# Autodesk Inventor assembly: Blue Alliance Arm
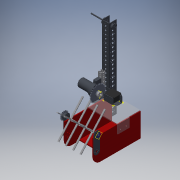
[picture p0: Inventor's stored thumbnail of the model, 180x180]
Saved by Autodesk Inventor 2016 (Build 200138000, 138)
## iProperties
Created: 2015-12-20
Part Number: Blue Alliance Arm
Document SubType Name: Assembly
Designer: tbloo
Author: tbloo
## Documents named in this file (14)
- C:\Users\TimB\Documents\GitHub\phi_robotics\3d-models\FTC_Tetrix_KOP_Block_Party\Tim Bloot Designs\JAr JaR Bot\Red Alliance Arm.iam
- C:\Users\TimB\Documents\GitHub\phi_robotics\3d-models\FTC_Tetrix_KOP_Block_Party\Tetrix_Kit_FTC\Autodesk Inventor Files\tetrix_axle.ipt
- C:\Users\TimB\Documents\GitHub\phi_robotics\3d-models\FTC_Tetrix_KOP_Block_Party\Tetrix_Kit_FTC\Autodesk Inventor Files\tetrix_axle_lock.iam
- C:\Users\TimB\Documents\GitHub\phi_robotics\3d-models\FTC_Tetrix_KOP_Block_Party\Tetrix_Kit_FTC\Autodesk Inventor Files\tetrix_c_channel-1.ipt
- C:\Users\TimB\Documents\GitHub\phi_robotics\3d-models\FTC_Tetrix_KOP_Block_Party\Tim Bloot Designs\JAr JaR Bot\cube channel short.ipt
- C:\Users\TimB\Documents\GitHub\phi_robotics\3d-models\FTC_Tetrix_KOP_Block_Party\Tetrix_Kit_FTC\Autodesk Inventor Files\tetrix_motor_mount-old.ipt
- C:\Users\TimB\Documents\GitHub\phi_robotics\3d-models\FTC_Tetrix_KOP_Block_Party\Tetrix_Kit_FTC\Autodesk Inventor Files\tetrix_motor.iam
- C:\Users\TimB\Documents\GitHub\phi_robotics\3d-models\FTC_Tetrix_KOP_Block_Party\Tetrix_Kit_FTC\Autodesk Inventor Files\tetrix_maxle_lock.iam
- C:\Users\TimB\Documents\GitHub\phi_robotics\3d-models\FTC_Tetrix_KOP_Block_Party\Tetrix_Kit_FTC\Autodesk Inventor Files\tetrix_chain_gear-32t.ipt
- C:\Users\TimB\Documents\GitHub\phi_robotics\3d-models\FTC_Tetrix_KOP_Block_Party\Tetrix_Kit_FTC\Autodesk Inventor Files\tetrix_screw.ipt
- C:\Users\TimB\Documents\GitHub\phi_robotics\3d-models\FTC_Tetrix_KOP_Block_Party\Tim Bloot Designs\JAr JaR Bot\Red Alliance Bucket.iam
- C:\Users\TimB\Documents\GitHub\phi_robotics\3d-models\FTC_Tetrix_KOP_Block_Party\Tetrix_Kit_FTC\Autodesk Inventor Files\tetrix_Lbracket-round.ipt
- C:\Users\TimB\Documents\GitHub\phi_robotics\3d-models\FTC_Tetrix_KOP_Block_Party\Tetrix_Kit_FTC\Autodesk Inventor Files\tetrix_c_channel-round.ipt
- C:\Users\TimB\Documents\GitHub\phi_robotics\3d-models\FTC_Tetrix_KOP_Block_Party\Tim Bloot Designs\JAr JaR Bot\cut c channel.ipt
## Components (16 placed, 13 different names)
1. tetrix_axle:1 — Rigid:1
2. tetrix_axle_lock:1 [sub-assembly] — Rigid:16
3. tetrix_axle_lock:2 [sub-assembly] — Rigid:1, Rigid:15
4. tetrix_c_channel-1:1 — Rigid:19
5. tetrix_c_channel-1:2 — Mate:1, Flush:1, Flush:2, Rigid:20
6. cube channel short:1 — Rigid:12, Rigid:17
7. tetrix_motor_mount-old:1 — Rigid:12, Rotational:1
8. tetrix_motor:1 [sub-assembly] — Rigid:11, Rotational:1
9. tetrix_maxle_lock:1 [sub-assembly] — Rigid:8, Rigid:11
10. tetrix_chain_gear-32t:1 — Rigid:8, Rigid:9, Rigid:10
11. tetrix_screw:1 — Rigid:10
12. tetrix_screw:2 — Rigid:9
13. Red Alliance Bucket:1 [sub-assembly] — Mate:1, Flush:1, Flush:2
14. tetrix_Lbracket-round:1 — Rigid:14, Rigid:18
15. tetrix_c_channel-round:1 — Rigid:14
16. cut c channel:1 — Rigid:15, Rigid:16, Rigid:17, Rigid:18, Rigid:19, Rigid:20
## Relationships (17: WeldJoint 13, Flush 2, RevoluteJoint 1, Mate 1)
- Rigid:1 [WeldJoint]: tetrix_axle:1 ↔ tetrix_axle_lock:2
- Rigid:8 [WeldJoint]: tetrix_maxle_lock:1 ↔ tetrix_chain_gear-32t:1
- Rigid:9 [WeldJoint]: tetrix_chain_gear-32t:1 ↔ tetrix_screw:2
- Rigid:10 [WeldJoint]: tetrix_chain_gear-32t:1 ↔ tetrix_screw:1
- Rigid:11 [WeldJoint] (-7 mm): tetrix_motor:1 ↔ tetrix_maxle_lock:1
- Rigid:12 [WeldJoint]: cube channel short:1 ↔ tetrix_motor_mount-old:1
- Rotational:1 [RevoluteJoint]: tetrix_motor_mount-old:1 ↔ tetrix_motor:1
- Mate:1: tetrix_c_channel-1:2 ↔ Red Alliance Bucket:1
- Flush:1: tetrix_c_channel-1:2 ↔ Red Alliance Bucket:1
- Flush:2: tetrix_c_channel-1:2 ↔ Red Alliance Bucket:1
- Rigid:14 [WeldJoint]: tetrix_Lbracket-round:1 ↔ tetrix_c_channel-round:1
- Rigid:15 [WeldJoint]: tetrix_axle_lock:2 ↔ cut c channel:1
- Rigid:16 [WeldJoint]: tetrix_axle_lock:1 ↔ cut c channel:1
- Rigid:17 [WeldJoint]: cube channel short:1 ↔ cut c channel:1
- Rigid:18 [WeldJoint]: tetrix_Lbracket-round:1 ↔ cut c channel:1
- Rigid:19 [WeldJoint]: tetrix_c_channel-1:1 ↔ cut c channel:1
- Rigid:20 [WeldJoint]: tetrix_c_channel-1:2 ↔ cut c channel:1
